# Autodesk Inventor assembly: Gimbal Assembly
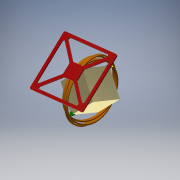
[picture p0: Inventor's stored thumbnail of the model, 180x180]
Saved by Autodesk Inventor 2018 (Build 220112000, 112)
## iProperties
Created: 2018-03-06
Part Number: Gimbal Assembly
Document SubType Name: Assembly
Designer: sterl
Author: sterl
## Documents named in this file (7)
- C:\Users\sterl\Documents\School\Slugsat\Gimbal\Gimbal Assembly.iam
- C:\Users\sterl\Documents\School\Slugsat\Gimbal\Cube.ipt
- C:\Users\sterl\Documents\School\Slugsat\Gimbal\Corners.ipt
- C:\Users\sterl\Documents\School\Slugsat\Gimbal\Inner.ipt
- C:\Users\sterl\Documents\School\Slugsat\Gimbal\Middle Ring.ipt
- C:\Users\sterl\Documents\School\Slugsat\Gimbal\Outer Ring.ipt
- C:\Users\sterl\Documents\School\Slugsat\Gimbal\Base.ipt
## Components (7 placed, 6 different names)
1. Cube:1 — Mate:1, Mate:2, Mate:3, Mate:4, Mate:5, Mate:6
2. Corners:1 — Mate:1, Mate:2, Mate:3, Mate:8
3. Corners:2 — Mate:4, Mate:5, Mate:6, Mate:7, Tangent:1
4. Inner:1 — Mate:7, Mate:8, Tangent:1, Mate:9, Mate:10, Tangent:2
5. Middle Ring:1 — Mate:9, Mate:10, Tangent:2, Mate:11, Mate:12, Tangent:3
6. Outer Ring:1 — Mate:11, Mate:12, Tangent:3, Mate:13, Mate:14, Mate:15
7. Base:1 — Mate:13, Mate:14, Mate:15
## Relationships (18: Mate 15, Tangent 3)
- Mate:1: Cube:1 ↔ Corners:1
- Mate:2: Cube:1 ↔ Corners:1
- Mate:3: Cube:1 ↔ Corners:1
- Mate:4: Cube:1 ↔ Corners:2
- Mate:5: Cube:1 ↔ Corners:2
- Mate:6: Cube:1 ↔ Corners:2
- Mate:7: Corners:2 ↔ Inner:1
- Mate:8: Corners:1 ↔ Inner:1
- Tangent:1: Corners:2 ↔ Inner:1
- Mate:9: Inner:1 ↔ Middle Ring:1
- Mate:10: Inner:1 ↔ Middle Ring:1
- Tangent:2: Inner:1 ↔ Middle Ring:1
- Mate:11: Middle Ring:1 ↔ Outer Ring:1
- Mate:12: Middle Ring:1 ↔ Outer Ring:1
- Tangent:3: Middle Ring:1 ↔ Outer Ring:1
- Mate:13: Outer Ring:1 ↔ Base:1
- Mate:14: Outer Ring:1 ↔ Base:1
- Mate:15: Outer Ring:1 ↔ Base:1
